# Autodesk Inventor assembly: shootingMechanism
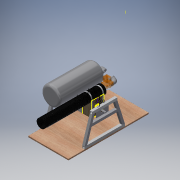
[picture p0: Inventor's stored thumbnail of the model, 180x180]
Saved by Autodesk Inventor 2017 (Build 210142000, 142)
## iProperties
Created: 2016-04-20
Part Number: shootingMechanism
Document SubType Name: Assembly
Designer: Administrator
Author: Administrator
## Documents named in this file (20)
- C:\Users\kingb\Documents\TShirty5\shootingMechanism.iam
- C:\Users\kingb\Documents\TShirty5\woodPlate.ipt
- C:\Users\kingb\Documents\TShirty5\daGasContiner.ipt
- C:\Users\kingb\Documents\TShirty5\16inSquarePipe.ipt
- C:\Users\kingb\Documents\TShirty5\10inSquarePipe.ipt
- C:\Users\kingb\Documents\TShirty5\Wonkey.ipt
- C:\Users\kingb\Documents\TShirty5\mountingPanelCannon.ipt
- C:\Users\kingb\Documents\TShirty5\midBrace.ipt
- C:\Users\kingb\Documents\TShirty5\bigShaft2.ipt
- C:\Users\kingb\Documents\TShirty5\Imported Components\Solenoid\Solenoid.ipt
- C:\Users\kingb\Documents\TShirty5\Cannon.ipt
- C:\Users\kingb\Documents\TShirty5\Cap.ipt
- C:\Users\kingb\Documents\TShirty5\CapSleeve.ipt
- C:\Users\kingb\Documents\TShirty5\Holder.ipt
- C:\Users\kingb\Documents\TShirty5\Strap.ipt
- C:\Users\kingb\Documents\TShirty5\Imported Components\Bolt4inch10-32\Bolt4inch10-32.ipt
- C:\Users\kingb\Documents\TShirty5\Imported Components\am-2568 500EX Hex Hub\am-2568 500EX Hex Hub.ipt
- C:\Users\kingb\Documents\TShirty5\Imported Components\1'2'HexBearing\1'2'HexBearing.ipt
- C:\Users\kingb\Documents\TShirty5\tankMount.ipt
- C:\Users\kingb\Documents\TShirty5\galvanizedIronElbowPipe.ipt
## Components (33 placed, 19 different names)
1. woodPlate:1 — Flush:1, Flush:6, Flush:7, Mate:5, Mate:13, Flush:32
2. daGasContiner:1 — Mate:60, Insert:5
3. 16inSquarePipe:3 — Mate:12, Mate:13, Mate:15, Flush:12, Mate:16, Flush:32
4. 16inSquarePipe:4 — Flush:8, Mate:5, Mate:6, Mate:8, Mate:9, Flush:11, Mate:18
5. 10inSquarePipe:1 — Flush:7, Flush:8, Mate:7, Flush:9, Mate:10, Mate:11, Flush:14, Flush:15, Mate:20, Flush:19, Flush:23, Flush:29, Angle:2
6. 10inSquarePipe:2 — Flush:6, Mate:14, Flush:13, Mate:17, Flush:14, Mate:19, Flush:16, Flush:22, Mate:21, Flush:26
7. Wonkey:1 — Mate:8, Mate:9, Flush:9
8. Wonkey:2 — Mate:16, Flush:13, Mate:17
9. Wonkey:3 — Flush:11, Mate:10, Mate:11, Mate:18, Flush:15, Mate:23, Flush:27
10. Wonkey:4 — Mate:12, Mate:14, Mate:15, Flush:12, Mate:19, Flush:16, Mate:22, Flush:24
11. mountingPanelCannon:2 — Mate:20, Flush:19, Flush:23, Flush:28, Flush:29, Mate:39, Mate:40
12. mountingPanelCannon:4 — Flush:22, Mate:21, Flush:25, Flush:26
13. midBrace:1 — Mate:23, Flush:27, Flush:28
14. midBrace:2 — Mate:22, Flush:24, Flush:25
15. bigShaft2:1 — Mate:41, Mate:42, Mate:56, Mate:57
16. Solenoid:1 — Insert:3, Angle:4, Insert:4
17. Cannon:1 — Insert:1, Mate:29, Mate:33, Mate:34
18. Cap:1 — Insert:1, Insert:2, Insert:3
19. CapSleeve:1 — Insert:2, Mate:30
20. Holder:1 — Mate:29, Mate:30, Mate:31, Mate:32, Flush:30, Flush:31, Mate:35, Mate:43, Angle:1, Mate:44, Mate:46, Angle:2, Flush:33, Angle:4
21. Strap:1 — Mate:32, Mate:33, Flush:31, Mate:58
22. Strap:2 — Mate:31, Mate:34, Flush:30, Mate:59
23. Bolt4inch10-32:1 — Mate:47, Mate:52
24. am-2568 500EX Hex Hub:2 — Mate:35, Mate:43, Angle:1, Mate:45, Mate:47, Mate:48, Mate:49, Mate:50, Mate:51, Mate:52, Mate:53, Mate:54, Mate:55, Mate:56, Mate:57
25. Bolt4inch10-32:2 — Mate:49, Mate:51
26. Bolt4inch10-32:3 — Mate:44, Mate:45
27. Bolt4inch10-32:4 — Mate:48, Mate:53
28. Bolt4inch10-32:5 — Mate:46, Mate:50
29. 1'2'HexBearing:1 — Mate:39, Mate:40, Mate:41, Mate:42
30. Bolt4inch10-32:6 — Mate:54, Mate:55
31. tankMount:1 — Mate:58, Flush:33, Mate:59, Mate:60
32. galvanizedIronElbowPipe:1 — Insert:5, Mate:61
33. galvanizedIronElbowPipe:2 — Insert:4, Mate:61
## Relationships (81: Mate 49, Flush 24, Insert 5, Angle 3)
- Flush:1 (190.5 mm): woodPlate:1
- Flush:6: woodPlate:1 ↔ 10inSquarePipe:2
- Flush:7: woodPlate:1 ↔ 10inSquarePipe:1
- Flush:8 (-76.2 mm): 16inSquarePipe:4 ↔ 10inSquarePipe:1
- Mate:5: woodPlate:1 ↔ 16inSquarePipe:4
- Mate:6: 16inSquarePipe:4
- Mate:7: 10inSquarePipe:1
- Mate:8: 16inSquarePipe:4 ↔ Wonkey:1
- Mate:9: 16inSquarePipe:4 ↔ Wonkey:1
- Flush:9: 10inSquarePipe:1 ↔ Wonkey:1
- Flush:11: 16inSquarePipe:4 ↔ Wonkey:3
- Mate:10: 10inSquarePipe:1 ↔ Wonkey:3
- Mate:11: 10inSquarePipe:1 ↔ Wonkey:3
- Mate:12: 16inSquarePipe:3 ↔ Wonkey:4
- Mate:13: woodPlate:1 ↔ 16inSquarePipe:3
- Mate:14: 10inSquarePipe:2 ↔ Wonkey:4
- Mate:15: 16inSquarePipe:3 ↔ Wonkey:4
- Flush:12: 16inSquarePipe:3 ↔ Wonkey:4
- Mate:16: 16inSquarePipe:3 ↔ Wonkey:2
- Flush:13: 10inSquarePipe:2 ↔ Wonkey:2
- Mate:17: 10inSquarePipe:2 ↔ Wonkey:2
- Flush:14: 10inSquarePipe:1 ↔ 10inSquarePipe:2
- Mate:18: 16inSquarePipe:4 ↔ Wonkey:3
- Flush:15: 10inSquarePipe:1 ↔ Wonkey:3
- Mate:19: 10inSquarePipe:2 ↔ Wonkey:4
- Flush:16: 10inSquarePipe:2 ↔ Wonkey:4
- Mate:20: 10inSquarePipe:1 ↔ mountingPanelCannon:2
- Flush:19 (63.5 mm): 10inSquarePipe:1 ↔ mountingPanelCannon:2
- Flush:22 (63.5 mm): 10inSquarePipe:2 ↔ mountingPanelCannon:4
- Mate:21: 10inSquarePipe:2 ↔ mountingPanelCannon:4
- Flush:23: 10inSquarePipe:1 ↔ mountingPanelCannon:2
- Mate:22: Wonkey:4 ↔ midBrace:2
- Flush:24: Wonkey:4 ↔ midBrace:2
- Flush:25: mountingPanelCannon:4 ↔ midBrace:2
- Flush:26: 10inSquarePipe:2 ↔ mountingPanelCannon:4
- Mate:23: Wonkey:3 ↔ midBrace:1
- Flush:27: Wonkey:3 ↔ midBrace:1
- Flush:28: mountingPanelCannon:2 ↔ midBrace:1
- Flush:29: 10inSquarePipe:1 ↔ mountingPanelCannon:2
- Insert:1: Cannon:1 ↔ Cap:1
- Insert:2: Cap:1 ↔ CapSleeve:1
- Insert:3: Solenoid:1 ↔ Cap:1
- Mate:29: Cannon:1 ↔ Holder:1
- Mate:30: CapSleeve:1 ↔ Holder:1
- Mate:31: Holder:1 ↔ Strap:2
- Mate:32: Holder:1 ↔ Strap:1
- Mate:33: Cannon:1 ↔ Strap:1
- Mate:34: Cannon:1 ↔ Strap:2
- Flush:30: Holder:1 ↔ Strap:2
- Flush:31: Holder:1 ↔ Strap:1
- Mate:35: Holder:1 ↔ am-2568 500EX Hex Hub:2
- Mate:39: mountingPanelCannon:2 ↔ 1'2'HexBearing:1
- Mate:40: mountingPanelCannon:2 ↔ 1'2'HexBearing:1
- Mate:41: bigShaft2:1 ↔ 1'2'HexBearing:1
- Mate:42: bigShaft2:1 ↔ 1'2'HexBearing:1
- Flush:32 (241.3 mm): woodPlate:1 ↔ 16inSquarePipe:3
- Mate:43: Holder:1 ↔ am-2568 500EX Hex Hub:2
- Angle:1 (0 deg): Holder:1 ↔ am-2568 500EX Hex Hub:2
- Mate:44: Holder:1 ↔ Bolt4inch10-32:3
- Mate:45: am-2568 500EX Hex Hub:2 ↔ Bolt4inch10-32:3
- Mate:46: Holder:1 ↔ Bolt4inch10-32:5
- Mate:47: Bolt4inch10-32:1 ↔ am-2568 500EX Hex Hub:2
- Mate:48: am-2568 500EX Hex Hub:2 ↔ Bolt4inch10-32:4
- Mate:49: am-2568 500EX Hex Hub:2 ↔ Bolt4inch10-32:2
- Mate:50: am-2568 500EX Hex Hub:2 ↔ Bolt4inch10-32:5
- Mate:51: am-2568 500EX Hex Hub:2 ↔ Bolt4inch10-32:2
- Mate:52: Bolt4inch10-32:1 ↔ am-2568 500EX Hex Hub:2
- Mate:53: am-2568 500EX Hex Hub:2 ↔ Bolt4inch10-32:4
- Mate:54: am-2568 500EX Hex Hub:2 ↔ Bolt4inch10-32:6
- Mate:55: am-2568 500EX Hex Hub:2 ↔ Bolt4inch10-32:6
- Angle:2 (0 deg): 10inSquarePipe:1 ↔ Holder:1
- Mate:56: bigShaft2:1 ↔ am-2568 500EX Hex Hub:2
- Mate:57: bigShaft2:1 ↔ am-2568 500EX Hex Hub:2
- Mate:58: Strap:1 ↔ tankMount:1
- Flush:33: Holder:1 ↔ tankMount:1
- Mate:59: Strap:2 ↔ tankMount:1
- Mate:60: daGasContiner:1 ↔ tankMount:1
- Angle:4 (0 deg): Solenoid:1 ↔ Holder:1
- Insert:4: Solenoid:1 ↔ galvanizedIronElbowPipe:2
- Insert:5: daGasContiner:1 ↔ galvanizedIronElbowPipe:1
- Mate:61: galvanizedIronElbowPipe:1 ↔ galvanizedIronElbowPipe:2
